# Autodesk Inventor assembly: Prusa_asm
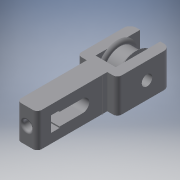
[picture p0: Inventor's stored thumbnail of the model, 180x180]
Saved by Autodesk Inventor 2019.3 (Build 233278000, 278)
## iProperties
Created: 2020-09-10
Part Number: Prusa_asm
Material: Generisch
Document SubType Name: Assembly
Designer: Nicolas Frick
Author: Nicolas Frick
## Documents named in this file (5)
- C:\Users\Nicolas Frick\Sync\OneDrive\airhockeybot\mechanical_design\inventor\Prusa\Prusa_asm.iam
- C:\Users\Nicolas Frick\Sync\OneDrive\airhockeybot\mechanical_design\inventor\Prusa\Prusa_clamp.ipt
- C:\Users\Nicolas Frick\Sync\OneDrive\airhockeybot\mechanical_design\inventor\Prusa\Prusa_pulley.ipt
- C:\Users\Nicolas Frick\Sync\OneDrive\airhockeybot\mechanical_design\inventor\Prusa\Distance.ipt
- C:\Users\Nicolas Frick\Sync\OneDrive\airhockeybot\mechanical_design\inventor\Prusa\624zz\snr_624zz_1.iam
## Components (5 placed, 4 different names)
1. Prusa_clamp:1 — Passend:6, Passend:7
2. Prusa_pulley:1 — Passend:1, Fluchtend:1, Passend:4, Passend:6
3. Distance:1 — Passend:2, Passend:3, Passend:7
4. snr_624zz_1:1 [sub-assembly] — Passend:1, Fluchtend:1, Passend:2, Passend:3, Passend:5
5. Distance:2 — Passend:4, Passend:5
## Relationships (8: Mate 7, Flush 1)
- Passend:1 [Mate]: Prusa_pulley:1 ↔ snr_624zz_1:1
- Fluchtend:1 [Flush] (1.9 mm): Prusa_pulley:1 ↔ snr_624zz_1:1
- Passend:2 [Mate]: Distance:1 ↔ snr_624zz_1:1
- Passend:3 [Mate]: Distance:1 ↔ snr_624zz_1:1
- Passend:4 [Mate]: Prusa_pulley:1 ↔ Distance:2
- Passend:5 [Mate]: snr_624zz_1:1 ↔ Distance:2
- Passend:6 [Mate]: Prusa_clamp:1 ↔ Prusa_pulley:1
- Passend:7 [Mate]: Prusa_clamp:1 ↔ Distance:1
